# Autodesk Inventor assembly: Assembly
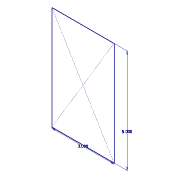
[picture p0: Inventor's stored thumbnail of the model, 180x180]
Saved by Autodesk Inventor 2015 SP1 (Build 190203100, 203)
## iProperties
RuleStatus: InUse
Created: 2015-06-24
Part Number: Assembly
Document SubType Name: Assembly
Designer: Derek
Author: Derek
## Documents named in this file (2)
- R:\WPT Drawings\CAD Drawings\Presses\Spirit\Spirit Inventor Files\Spirit [Site] - Inventor Files\Assembly.iam
- R:\WPT Drawings\CAD Drawings\Presses\Spirit\Spirit Inventor Files\Spirit [Site] - Inventor Files\Sketch Part.ipt
## Components (1 placed, 1 different names)
1. Sketch Part:1
## Named parameters: Width = 76.2 mm, Height = 127 mm
